# Autodesk Inventor assembly: 90_Degree_and_180_Degree
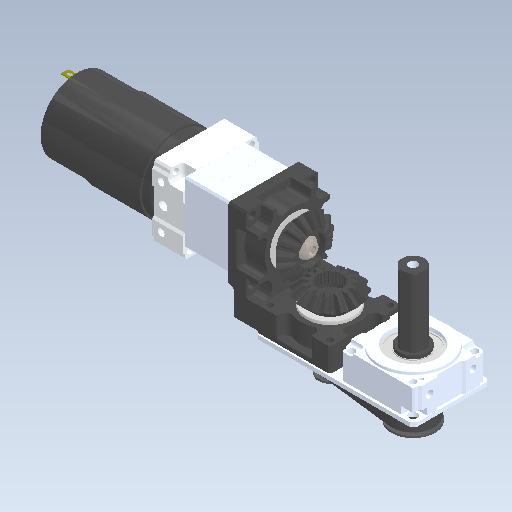
[picture p0: Inventor's stored thumbnail of the model, 512x512]
Saved by Autodesk Inventor 2020 (Build 240168000, 168)
## iProperties
Created: 2018-09-07
Part Number: 90_Degree_and_180_Degree
Description: STEP AP214
Document SubType Name: Assembly
Designer: Collin
Sending System: SolidWorks 2017
Preprocessor: SwSTEP 2.0
Title: 90 Degree and 180.STEP
Revision Number: ANY
## Documents named in this file (13)
- D:\My Docs\Robotics\Robot Stuff\STEP Files\VPs\90 Degree and 180 Degree VP\90_Degree_and_180_Degree.iam
- D:\My Docs\Robotics\Robot Stuff\STEP Files\VPs\90 Degree and 180 Degree VP\217-6293-000 Rev1.iam
- D:\My Docs\Robotics\Robot Stuff\STEP Files\VPs\90 Degree and 180 Degree VP\217-6043-001 Rev4.ipt
- D:\My Docs\Robotics\Robot Stuff\STEP Files\VPs\90 Degree and 180 Degree VP\GT2 12 24 Belt.ipt
- D:\My Docs\Robotics\Robot Stuff\STEP Files\VPs\90 Degree and 180 Degree VP\217-5871-001 Rev4.ipt
- D:\My Docs\Robotics\Robot Stuff\STEP Files\VPs\90 Degree and 180 Degree VP\217-5875-001 Rev3.ipt
- D:\My Docs\Robotics\Robot Stuff\STEP Files\VPs\90 Degree and 180 Degree VP\VersaPlanetary Output Shafts_0.500_ Hex (217-2615-003).iam
- D:\My Docs\Robotics\Robot Stuff\STEP Files\VPs\90 Degree and 180 Degree VP\VersaPlanetary v2 Output Block.iam
- D:\My Docs\Robotics\Robot Stuff\STEP Files\VPs\90 Degree and 180 Degree VP\#.25-20 BHS, Grade 8 Steel Rev1_SBS2520-0375BO.ipt
- D:\My Docs\Robotics\Robot Stuff\STEP Files\VPs\90 Degree and 180 Degree VP\217-6293-006 Rev1.ipt
- D:\My Docs\Robotics\Robot Stuff\STEP Files\VPs\2 Stage VP with 775pro\217-2625-025 Rev1.ipt
- D:\My Docs\Robotics\Robot Stuff\STEP Files\VPs\90 Degree and 180 Degree VP\217-2816-001 Rev1.ipt
- D:\My Docs\Robotics\Robot Stuff\STEP Files\VPs\2 Stage VP with 775pro\775pro_217-4347.ipt
## Components (13 placed, 12 different names)
1. 217-6043-001 Rev4_3 — Mate:3, Mate:4, Mate:5, Mate:8, Mate:9, Angle:1
2. GT2 12 24 Belt_4
3. 217-5871-001 Rev4_5
4. 217-5875-001 Rev3_6 — Mate:6, Mate:7
5. #.25-20 BHS, Grade 8 Steel Rev1_SBS2520-0375BO_19
6. 217-6293-006 Rev1_20
7. VersaPlanetary v2 Output Block:1 [sub-assembly] — Mate:1, Mate:2, Mate:3, Mate:4, Mate:5
8. VersaPlanetary Output Shafts_0.500_ Hex (217-2615-003):1 [sub-assembly] — Mate:1, Mate:2, Mate:6, Mate:7
9. 217-6293-000 Rev1:1 [sub-assembly] — Mate:8, Mate:9, Angle:1, Mate:10, Mate:11, Mate:15
10. 217-2625-025 Rev1:1 — Mate:14, Mate:15, Mate:16, Mate:17
11. 217-2816-001 Rev1:1 — Mate:12, Mate:13, Mate:14
12. 217-2816-001 Rev1:2 — Mate:10, Mate:11, Mate:12, Mate:13
13. 775pro_217-4347:1 — Mate:16, Mate:17
## Relationships (18: Mate 17, Angle 1)
- Mate:1: VersaPlanetary v2 Output Block:1 ↔ VersaPlanetary Output Shafts_0.500_ Hex (217-2615-003):1
- Mate:2: VersaPlanetary v2 Output Block:1 ↔ VersaPlanetary Output Shafts_0.500_ Hex (217-2615-003):1
- Mate:3: 217-6043-001 Rev4_3 ↔ VersaPlanetary v2 Output Block:1
- Mate:4: 217-6043-001 Rev4_3 ↔ VersaPlanetary v2 Output Block:1
- Mate:5: 217-6043-001 Rev4_3 ↔ VersaPlanetary v2 Output Block:1
- Mate:6: 217-5875-001 Rev3_6 ↔ VersaPlanetary Output Shafts_0.500_ Hex (217-2615-003):1
- Mate:7: 217-5875-001 Rev3_6 ↔ VersaPlanetary Output Shafts_0.500_ Hex (217-2615-003):1
- Mate:8: 217-6043-001 Rev4_3 ↔ 217-6293-000 Rev1:1
- Mate:9: 217-6043-001 Rev4_3 ↔ 217-6293-000 Rev1:1
- Angle:1 (0 deg): 217-6043-001 Rev4_3 ↔ 217-6293-000 Rev1:1
- Mate:10: 217-6293-000 Rev1:1 ↔ 217-2816-001 Rev1:2
- Mate:11: 217-6293-000 Rev1:1 ↔ 217-2816-001 Rev1:2
- Mate:12: 217-2816-001 Rev1:1 ↔ 217-2816-001 Rev1:2
- Mate:13: 217-2816-001 Rev1:1 ↔ 217-2816-001 Rev1:2
- Mate:14: 217-2625-025 Rev1:1 ↔ 217-2816-001 Rev1:1
- Mate:15: 217-6293-000 Rev1:1 ↔ 217-2625-025 Rev1:1
- Mate:16: 217-2625-025 Rev1:1 ↔ 775pro_217-4347:1
- Mate:17: 217-2625-025 Rev1:1 ↔ 775pro_217-4347:1
